# Autodesk Inventor assembly: Gantry
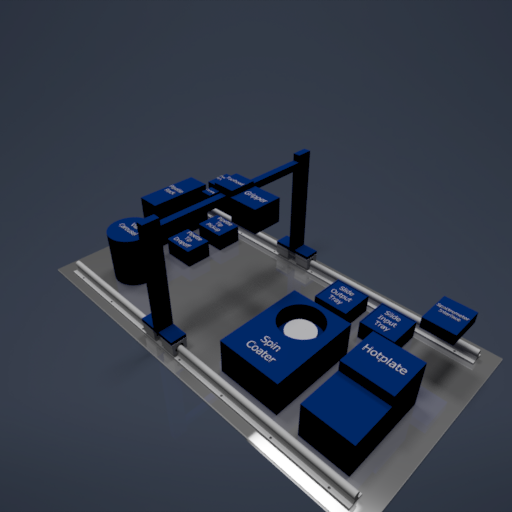
[picture p0: Inventor's stored thumbnail of the model, 512x512]
Saved by Autodesk Inventor 2025.1 (Build 291241000, 241)
## iProperties
Created: 2024-10-31
Part Number: Gantry
Document SubType Name: Assembly
Designer: jerem
Author: jerem
## Documents named in this file (14)
- C:\Users\jerem\Documents\GitHub\Perovskite-Automated-Synthesis-System\CAD\Gantry\Gantry.iam
- C:\Users\jerem\Documents\GitHub\Perovskite-Automated-Synthesis-System\CAD\Non 3D Printed Parts\Base Plate.ipt
- C:\Users\jerem\Documents\GitHub\Perovskite-Automated-Synthesis-System\CAD\Non 3D Printed Parts\Linear Rails\Linear Rail.ipt
- C:\Users\jerem\Documents\GitHub\Perovskite-Automated-Synthesis-System\CAD\Non 3D Printed Parts\Linear Rails\Linear Rail Slider Block.ipt
- C:\Users\jerem\Documents\GitHub\Perovskite-Automated-Synthesis-System\CAD\Non 3D Printed Parts\Objects\HotPlate.ipt
- C:\Users\jerem\Documents\GitHub\Perovskite-Automated-Synthesis-System\CAD\Non 3D Printed Parts\Objects\VialCarousel.ipt
- C:\Users\jerem\Documents\GitHub\Perovskite-Automated-Synthesis-System\CAD\Non 3D Printed Parts\Objects\TipPickup.ipt
- C:\Users\jerem\Documents\GitHub\Perovskite-Automated-Synthesis-System\CAD\Non 3D Printed Parts\Objects\TipDropoff.ipt
- C:\Users\jerem\Documents\GitHub\Perovskite-Automated-Synthesis-System\CAD\Non 3D Printed Parts\Objects\SpinCoater.ipt
- C:\Users\jerem\Documents\GitHub\Perovskite-Automated-Synthesis-System\CAD\Non 3D Printed Parts\Objects\SpectrometerMeasurer.ipt
- C:\Users\jerem\Documents\GitHub\Perovskite-Automated-Synthesis-System\CAD\Non 3D Printed Parts\Objects\Slide Output Tray.ipt
- C:\Users\jerem\Documents\GitHub\Perovskite-Automated-Synthesis-System\CAD\Non 3D Printed Parts\Objects\Slide Input Tray.ipt
- C:\Users\jerem\Documents\GitHub\Perovskite-Automated-Synthesis-System\CAD\Non 3D Printed Parts\Objects\PipetteRack.ipt
- C:\Users\jerem\Documents\GitHub\Perovskite-Automated-Synthesis-System\CAD\Non 3D Printed Parts\Objects\ToolheadMock.ipt
## Components (17 placed, 13 different names)
1. Base Plate:1 — Flush:1, Flush:2, Mate:1, Mate:2, Angle:1, Angle:2, Angle:3, Angle:4, Mate:8, Mate:9, Mate:10, Mate:11, Mate:12, Angle:5, Mate:13, Mate:14, Mate:15
2. Linear Rail:1 — Flush:1, Flush:2, Mate:1, Flush:3, Mate:3, Mate:4, Mate:5
3. Linear Rail:2 — Mate:2, Flush:3, Mate:3, Mate:6, Mate:7
4. Linear Rail Slider Block:1 — Mate:4, Angle:4, Flush:4, Mate:16
5. Linear Rail Slider Block:2 — Mate:5, Angle:3, Flush:5, Mate:16
6. Linear Rail Slider Block:3 — Mate:6, Angle:1, Flush:5, Flush:6, Flush:7
7. Linear Rail Slider Block:4 — Mate:7, Angle:2, Flush:4, Mate:17
8. HotPlate:1 — Mate:8
9. VialCarousel:1 — Mate:11
10. TipPickup:1 — Mate:9
11. TipDropoff:1 — Mate:10
12. SpinCoater:1 — Mate:12, Angle:5
13. SpectrometerMeasurer:1
14. Slide Output Tray:1 — Mate:13
15. Slide Input Tray:1 — Mate:14
16. PipetteRack:1 — Mate:15
17. ToolheadMock:1 — Mate:17, Flush:6, Flush:7
## Relationships (29: Mate 17, Flush 7, Angle 5)
- Flush:1 (50 mm): Base Plate:1 ↔ Linear Rail:1
- Flush:2 (25 mm): Base Plate:1 ↔ Linear Rail:1
- Mate:1: Base Plate:1 ↔ Linear Rail:1
- Mate:2: Base Plate:1 ↔ Linear Rail:2
- Flush:3: Linear Rail:1 ↔ Linear Rail:2
- Mate:3 (450 mm): Linear Rail:1 ↔ Linear Rail:2
- Mate:4: Linear Rail:1 ↔ Linear Rail Slider Block:1
- Mate:5: Linear Rail:1 ↔ Linear Rail Slider Block:2
- Mate:6: Linear Rail:2 ↔ Linear Rail Slider Block:3
- Mate:7: Linear Rail:2 ↔ Linear Rail Slider Block:4
- Angle:1 (0 deg): Base Plate:1 ↔ Linear Rail Slider Block:3
- Angle:2 (0 deg): Base Plate:1 ↔ Linear Rail Slider Block:4
- Angle:3 (0 deg): Base Plate:1 ↔ Linear Rail Slider Block:2
- Angle:4 (0 deg): Base Plate:1 ↔ Linear Rail Slider Block:1
- Flush:4: Linear Rail Slider Block:1 ↔ Linear Rail Slider Block:4
- Flush:5: Linear Rail Slider Block:2 ↔ Linear Rail Slider Block:3
- Mate:8: Base Plate:1 ↔ HotPlate:1
- Mate:9: Base Plate:1 ↔ TipPickup:1
- Mate:10: Base Plate:1 ↔ TipDropoff:1
- Mate:11: Base Plate:1 ↔ VialCarousel:1
- Mate:12: Base Plate:1 ↔ SpinCoater:1
- Angle:5 (0 deg): Base Plate:1 ↔ SpinCoater:1
- Mate:13: Base Plate:1 ↔ Slide Output Tray:1
- Mate:14: Base Plate:1 ↔ Slide Input Tray:1
- Mate:15: Base Plate:1 ↔ PipetteRack:1
- Mate:16 (30 mm): Linear Rail Slider Block:1 ↔ Linear Rail Slider Block:2
- Mate:17: Linear Rail Slider Block:4 ↔ ToolheadMock:1
- Flush:6: Linear Rail Slider Block:3 ↔ ToolheadMock:1
- Flush:7: Linear Rail Slider Block:3 ↔ ToolheadMock:1
